# Autodesk Inventor assembly: 轮腿
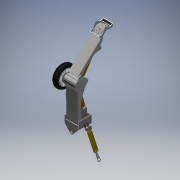
[picture p0: Inventor's stored thumbnail of the model, 180x180]
Saved by Autodesk Inventor 2019 (Build 230136000, 136)
## iProperties
Created: 2018-12-12
Part Number: 轮腿
Document SubType Name: Assembly
Designer: Administrator
Author: Administrator
## Documents named in this file (16)
- C:\Users\Administrator\Desktop\机械产品数字化设计大赛\轮腿\右轮腿.iam
- C:\Users\Administrator\Desktop\机械产品数字化设计大赛\轮腿\底座.ipt
- C:\Users\Administrator\Desktop\机械产品数字化设计大赛\轮腿\一级外壳左.ipt
- C:\Users\Administrator\Desktop\机械产品数字化设计大赛\轮腿\销钉400_60 .ipt
- C:\Users\Administrator\Desktop\机械产品数字化设计大赛\轮腿\液压杆体.ipt
- C:\Users\Administrator\Desktop\机械产品数字化设计大赛\轮腿\液压杆.ipt
- C:\Users\Administrator\Desktop\机械产品数字化设计大赛\轮腿\销钉340_54.ipt
- C:\Users\Administrator\Desktop\机械产品数字化设计大赛\轮腿\销钉120_60.ipt
- C:\Users\Administrator\Desktop\机械产品数字化设计大赛\轮腿\二级外壳.ipt
- C:\Users\Administrator\Desktop\机械产品数字化设计大赛\轮腿\销钉340_50.ipt
- C:\Users\Administrator\Desktop\机械产品数字化设计大赛\轮腿\末端爪.ipt
- C:\Users\Administrator\Desktop\机械产品数字化设计大赛\轮腿\末端销钉120_40.ipt
- C:\Users\Administrator\Desktop\机械产品数字化设计大赛\轮腿\销钉340_60.ipt
- C:\Users\Administrator\Desktop\机械产品数字化设计大赛\轮腿\销钉280_54.ipt
- C:\Users\Administrator\Desktop\机械产品数字化设计大赛\轮腿\轮子\HP2 Raceparts Complette Tyre.iam
- C:\Users\Administrator\Desktop\机械产品数字化设计大赛\轮腿\液压杆盖.ipt
## Components (22 placed, 15 different names)
1. 底座:1 — 插入:1, 配合:3, 配合:4, 配合:6, 配合:12, 配合:13, 配合:21, 配合:22, 配合:41, 配合:42
2. 销钉400_60 :1 — 插入:1, 配合:5
3. 液压杆体:1 — 配合:3, 配合:4, 配合:7, 插入:3, 配合:39
4. 一级外壳左:1 — 配合:5, 配合:6, 配合:9, 配合:10, 表面齐平:1, 配合:15, 配合:16, 配合:24, 配合:25, 配合:34, 配合:35, 配合:38
5. 液压杆:1 — 配合:7, 配合:11, 配合:39
6. 销钉340_54:1 — 配合:9, 配合:10, 配合:11
7. 销钉120_60:1 — 配合:12, 配合:13
8. 二级外壳:1 — 表面齐平:1, 配合:26, 配合:27, 配合:28, 配合:30, 配合:31, 配合:32, 配合:33, 配合:36, 配合:37
9. 销钉340_50:1 — 配合:15, 配合:16, 配合:26
10. 末端爪:1 — 配合:30, 配合:31
11. 末端销钉120_40:1 — 配合:32, 配合:33
12. 液压杆体:2 — 配合:21, 配合:22, 配合:23, 插入:2
13. 液压杆:2 — 配合:23
14. 液压杆体:3 — 配合:24, 配合:25, 配合:29, 插入:4, 配合:40
15. 液压杆:3 — 配合:27, 配合:28, 配合:29, 配合:40
16. 销钉340_60:1 — 配合:34, 配合:35
17. 销钉280_54:1 — 配合:36, 配合:37
18. HP2 Raceparts Complette Tyre:1 [sub-assembly] — 配合:38
19. 液压杆盖:1 — 插入:2
20. 液压杆盖:2 — 插入:3
21. 液压杆盖:3 — 插入:4
22. 销钉120_60:2 — 配合:41, 配合:42
## Relationships (39: Mate 34, Insert 4, Flush 1)
- 插入:1 [Insert]: 底座:1 ↔ 销钉400_60 :1
- 配合:3 [Mate]: 底座:1 ↔ 液压杆体:1
- 配合:4 [Mate]: 底座:1 ↔ 液压杆体:1
- 配合:5 [Mate]: 销钉400_60 :1 ↔ 一级外壳左:1
- 配合:6 [Mate] (10 mm): 底座:1 ↔ 一级外壳左:1
- 配合:7 [Mate]: 液压杆体:1 ↔ 液压杆:1
- 配合:9 [Mate]: 一级外壳左:1 ↔ 销钉340_54:1
- 配合:10 [Mate]: 一级外壳左:1 ↔ 销钉340_54:1
- 配合:11 [Mate]: 液压杆:1 ↔ 销钉340_54:1
- 配合:12 [Mate]: 底座:1 ↔ 销钉120_60:1
- 配合:13 [Mate]: 底座:1 ↔ 销钉120_60:1
- 表面齐平:1 [Flush] (30 mm): 一级外壳左:1 ↔ 二级外壳:1
- 配合:15 [Mate]: 一级外壳左:1 ↔ 销钉340_50:1
- 配合:16 [Mate]: 一级外壳左:1 ↔ 销钉340_50:1
- 配合:21 [Mate]: 底座:1 ↔ 液压杆体:2
- 配合:22 [Mate]: 底座:1 ↔ 液压杆体:2
- 配合:23 [Mate]: 液压杆体:2 ↔ 液压杆:2
- 配合:24 [Mate]: 一级外壳左:1 ↔ 液压杆体:3
- 配合:25 [Mate]: 一级外壳左:1 ↔ 液压杆体:3
- 配合:26 [Mate]: 二级外壳:1 ↔ 销钉340_50:1
- 配合:27 [Mate]: 二级外壳:1 ↔ 液压杆:3
- 配合:28 [Mate]: 二级外壳:1 ↔ 液压杆:3
- 配合:29 [Mate]: 液压杆体:3 ↔ 液压杆:3
- 配合:30 [Mate]: 二级外壳:1 ↔ 末端爪:1
- 配合:31 [Mate]: 二级外壳:1 ↔ 末端爪:1
- 配合:32 [Mate]: 二级外壳:1 ↔ 末端销钉120_40:1
- 配合:33 [Mate]: 二级外壳:1 ↔ 末端销钉120_40:1
- 配合:34 [Mate]: 一级外壳左:1 ↔ 销钉340_60:1
- 配合:35 [Mate]: 一级外壳左:1 ↔ 销钉340_60:1
- 配合:36 [Mate]: 二级外壳:1 ↔ 销钉280_54:1
- 配合:37 [Mate]: 二级外壳:1 ↔ 销钉280_54:1
- 配合:38 [Mate]: 一级外壳左:1 ↔ HP2 Raceparts Complette Tyre:1
- 插入:2 [Insert]: 液压杆体:2 ↔ 液压杆盖:1
- 插入:3 [Insert]: 液压杆体:1 ↔ 液压杆盖:2
- 插入:4 [Insert]: 液压杆体:3 ↔ 液压杆盖:3
- 配合:39 [Mate]: 液压杆体:1 ↔ 液压杆:1
- 配合:40 [Mate]: 液压杆体:3 ↔ 液压杆:3
- 配合:41 [Mate]: 底座:1 ↔ 销钉120_60:2
- 配合:42 [Mate]: 底座:1 ↔ 销钉120_60:2
